# Autodesk Inventor assembly: A_Airbert
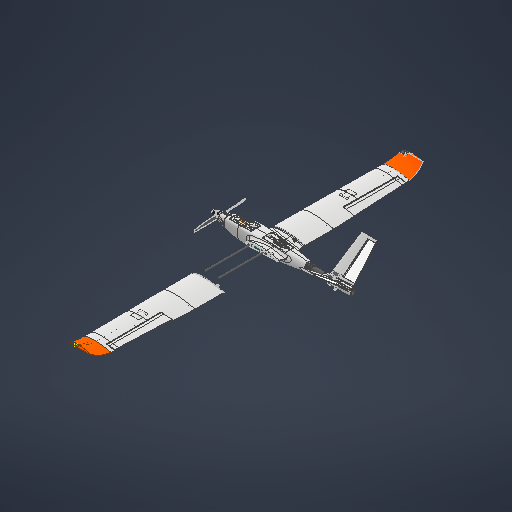
[picture p0: Inventor's stored thumbnail of the model, 512x512]
Saved by Autodesk Inventor 2026.2 (Build 302298000, 298)
## iProperties
Created: 2025-08-22
Part Number: A_Airbert
Document SubType Name: Assembly
Designer: FAL
Mass: 940.749 g
Surface Area: 6231.37 cm^2
Volume: 1491.38 cm^3
Author: FAL
## Documents named in this file (6)
- C:\Users\FAL\git\AIRBERT\CAD\A_Airbert.iam
- C:\Users\FAL\git\AIRBERT\CAD\Wing\A_Wing.iam
- C:\Users\FAL\git\AIRBERT\CAD\Fuselage\A_Fuselage.iam
- C:\Users\FAL\git\AIRBERT\CAD\Aft\A_Aft.iam
- C:\Users\FAL\git\AIRBERT\CAD\alternativeWing\CAD\Wing\A_Wing.iam
- C:\Users\FAL\git\AIRBERT\CAD\Wing\mirror\A_Wing_MIR.iam
## Components (5 placed, 4 different names)
1. A_Wing:1 [sub-assembly] — Fluchtend:1, Fluchtend:2, Fluchtend:3
2. A_Wing:2 [sub-assembly] — Fluchtend:10, Fluchtend:11, Fluchtend:12
3. A_Fuselage:1 [sub-assembly] — Fluchtend:4, Fluchtend:5, Fluchtend:6
4. A_Aft:1 [sub-assembly] — Fluchtend:7, Fluchtend:8, Fluchtend:9
5. A_Wing_MIR:1 [sub-assembly] — Passend:1, Passend:2, Fluchtend:13
## Relationships (15: Flush 13, Mate 2)
- Fluchtend:1 [Flush]: A_Wing:1
- Fluchtend:2 [Flush]: A_Wing:1
- Fluchtend:3 [Flush]: A_Wing:1
- Fluchtend:4 [Flush]: A_Fuselage:1
- Fluchtend:5 [Flush]: A_Fuselage:1
- Fluchtend:6 [Flush]: A_Fuselage:1
- Fluchtend:7 [Flush]: A_Aft:1
- Fluchtend:8 [Flush]: A_Aft:1
- Fluchtend:9 [Flush]: A_Aft:1
- Fluchtend:10 [Flush]: A_Wing:2
- Fluchtend:11 [Flush]: A_Wing:2
- Fluchtend:12 [Flush]: A_Wing:2
- Passend:1 [Mate]: A_Wing_MIR:1
- Passend:2 [Mate]: A_Wing_MIR:1
- Fluchtend:13 [Flush]: A_Wing_MIR:1
